# Autodesk Inventor assembly: case_assembly
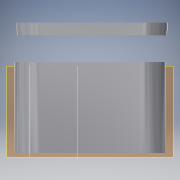
[picture p0: Inventor's stored thumbnail of the model, 180x180]
Saved by Autodesk Inventor 2019 (Build 230136000, 136)
## iProperties
Created: 2019-01-02
Part Number: case_assembly
Document SubType Name: Assembly
Designer: jmc
Author: jmc
## Documents named in this file (9)
- D:\Inventor\Projects\CatFeeder\version2 (fixed enclosure)\version2.iam
- D:\Inventor\Projects\CatFeeder\Case\version2\case.ipt
- D:\Inventor\Projects\3party\Boards\ArduinoNano\arduino nano.iam
- D:\Inventor\Projects\3party\Boards\Raspberry Pi 3\Raspberry Pi 3.ipt
- D:\Inventor\Projects\3party\Trasformer\Transformer.ipt
- D:\Inventor\Projects\CatFeeder\Case\version2\case_top.ipt
- D:\Inventor\Projects\CatFeeder\Case\version2\case_bottom.ipt
- D:\Inventor\Projects\CatFeeder\Case\version2\Pata.ipt
- D:\Inventor\Projects\CatFeeder\Case\version2\pata_macho.ipt
## Components (14 placed, 8 different names)
1. case:1
2. case_top:1 — Rigid:9
3. case_bottom:1 — Rigid:1, Rigid:3, Rigid:4, Flush:1, Rotational:1, Rigid:6, Rigid:7, Rigid:8, Rigid:9
4. arduino nano:1 [sub-assembly] — Rigid:4
5. Raspberry Pi 3:1 — Rigid:1
6. Transformer:1 — Rigid:3
7. pata_macho:4 — Rotational:5
8. pata_macho:3 — Rotational:3
9. pata_macho:2 — Rotational:4
10. pata_macho:1 — Rotational:2
11. Pata:1 — Flush:1, Rotational:1, Rotational:2
12. Pata:2 — Rigid:8, Rotational:5
13. Pata:3 — Rigid:7, Rotational:3
14. Pata:4 — Rigid:6, Rotational:4
## Relationships (13: WeldJoint 7, RevoluteJoint 5, Flush 1)
- Rigid:1 [WeldJoint]: case_bottom:1 ↔ Raspberry Pi 3:1
- Rigid:3 [WeldJoint]: case_bottom:1 ↔ Transformer:1
- Rigid:4 [WeldJoint]: case_bottom:1 ↔ arduino nano:1
- Flush:1: case_bottom:1 ↔ Pata:1
- Rotational:1 [RevoluteJoint]: case_bottom:1 ↔ Pata:1
- Rigid:6 [WeldJoint]: case_bottom:1 ↔ Pata:4
- Rigid:7 [WeldJoint]: case_bottom:1 ↔ Pata:3
- Rigid:8 [WeldJoint]: case_bottom:1 ↔ Pata:2
- Rotational:2 [RevoluteJoint]: pata_macho:1 ↔ Pata:1
- Rotational:3 [RevoluteJoint]: pata_macho:3 ↔ Pata:3
- Rotational:4 [RevoluteJoint]: pata_macho:2 ↔ Pata:4
- Rotational:5 [RevoluteJoint]: pata_macho:4 ↔ Pata:2
- Rigid:9 [WeldJoint]: case_top:1 ↔ case_bottom:1
